# Autodesk Inventor assembly: Main Assembly
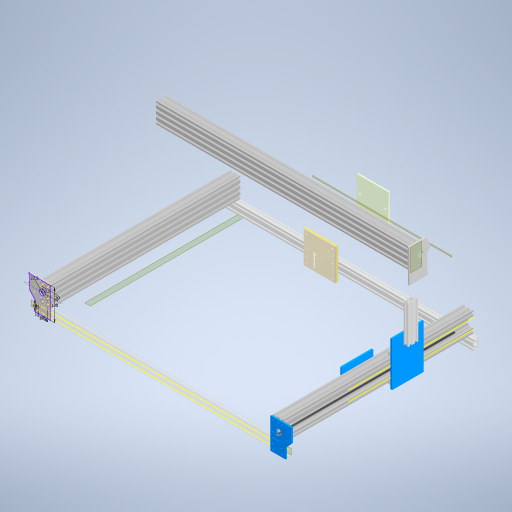
[picture p0: Inventor's stored thumbnail of the model, 512x512]
Saved by Autodesk Inventor 2023.2 (Build 272271000, 271)
## iProperties
Created: 2023-01-31
Part Number: Main Assembly
Document SubType Name: Assembly
Designer: dmargari
Mass: 176937 g
Surface Area: 89724.7 cm^2
Volume: 174359 cm^3
Density: 1.01479 g/cm^3
Author: dmargari
## iProperties of the stored document Solid-V-Xtreme-Wheel.ipt
Created: 2015-07-29
Part Number: Xtreme Solid V Wheel
Material: Generic
Description: STEP AP203
Document SubType Name: Modeling
Designer: dmargari
Density: 1 g/cm^3
Appearance: Default
Mass: 2.24603 g
Surface Area: 16.605 cm^2
Volume: 2.24603 cm^3
Sending System: SolidWorks 2014
Preprocessor: SwSTEP 2.0
Title: Xtreme Solid V Wheel.step
Revision Number: ANY
## iProperties of the stored document ACME-Nut-Block.ipt
Created: 2015-07-29
Part Number: 8mm Acme Nut Block
Material: Generic
Description: STEP AP203
Document SubType Name: Modeling
Designer: dmargari
Density: 1 g/cm^3
Appearance: Default
Sending System: SolidWorks 2014
Preprocessor: SwSTEP 2.0
Title: 8mm Acme Nut Block.step
Revision Number: ANY
## Documents named in this file (18)
- \\icnas3.cc.ic.ac.uk\dmargari\Inventor\Autosampler V3\Main Assembly.iam
- \\icnas3.cc.ic.ac.uk\dmargari\Inventor\Autosampler V3\Desk.ipt
- **\\icnas3.cc.ic.ac.uk\dmargari\Inventor\Autosampler V3\Main Assembly.iam*LocalDocs*xAaaaaibaAaaaaaaaAaaaapz5Ha*Solid-V-Xtreme-Wheel.ipt
- \\icnas3.cc.ic.ac.uk\dmargari\Inventor\Autosampler V3\C beam gantry (small side y axis).ipt
- \\icnas3.cc.ic.ac.uk\dmargari\Inventor\Autosampler V3\C beam gantry (big side y axis).ipt
- \\icnas3.cc.ic.ac.uk\dmargari\Inventor\Content Center Files\R2023\en-US\20x40\1000.ipt
- \\icnas3.cc.ic.ac.uk\dmargari\Inventor\Content Center Files\R2023\en-US\C beam extrusion\250.ipt
- **\\icnas3.cc.ic.ac.uk\dmargari\Inventor\Autosampler V3\Main Assembly.iam*LocalDocs*xAaaaaqaaAaaaaaaaAaaaqjz0Qe*ACME-Nut-Block.ipt
- \\icnas3.cc.ic.ac.uk\dmargari\Inventor\Autosampler V3\lead screw 8mm 700mm.ipt
- \\icnas3.cc.ic.ac.uk\dmargari\Inventor\Autosampler V3\Y axis motor mount new.ipt
- \\icnas3.cc.ic.ac.uk\dmargari\Inventor\Autosampler V3\X axis motor mount.ipt
- \\icnas3.cc.ic.ac.uk\dmargari\Inventor\Autosampler V3\20x40 extrusion x axis.ipt
- \\icnas3.cc.ic.ac.uk\dmargari\Inventor\Content Center Files\R2023\en-US\C beam extrusion\500.ipt
- \\icnas3.cc.ic.ac.uk\dmargari\Inventor\Autosampler V3\X axis carriage.ipt
- \\icnas3.cc.ic.ac.uk\dmargari\Inventor\Autosampler V3\X axis carriage small.ipt
- \\icnas3.cc.ic.ac.uk\dmargari\Inventor\Autosampler V3\X axis carriage small side.ipt
- \\icnas3.cc.ic.ac.uk\dmargari\Inventor\Autosampler V3\3rd-party-models\Solid-V-Xtreme-Wheel\Solid-V-Xtreme-Wheel.step
- \\icnas3.cc.ic.ac.uk\dmargari\Inventor\Autosampler V3\3rd-party-models\Ooznest-ACME-Nut-Block\ACME-Nut-Block.step
## Components (20 placed, 15 different names)
1. Desk:1 — Flush:2, Mate:31, Flush:44, Flush:45, Mate:32, Flush:47
2. C beam extrusion 250:1
3. C beam extrusion 250:2 — Flush:57
4. C beam gantry (small side y axis):1
5. C beam gantry (big side y axis):1 — Flush:57, Mate:34, Flush:50, Mate:35, Flush:51, Flush:52, Flush:58, Mate:42, Rigid:23
6. 20x40 extrusion x axis:1 — Mate:42, Rigid:23, Mate:43
7. 20x40 1000:1 — Mate:31, Flush:44, Flush:45, Mate:33, Mate:38, Flush:55, Flush:56
8. 20x40 1000:2 — Mate:32, Flush:47, Mate:33
9. ACME-Nut-Block:1 — Mate:34, Flush:50, Flush:58
10. ACME-Nut-Block:2 — Mate:35, Flush:51, Flush:52, Mate:36
11. lead screw 8mm 700mm:1 — Mate:36
12. Y axis motor mount new:1
13. Y axis motor mount new:2 — Mate:38, Flush:55, Flush:56
14. Solid-V-Xtreme-Wheel:9
15. Solid-V-Xtreme-Wheel:10
16. X axis motor mount:1 — Rotational:11, Mate:43
17. C beam extrusion 500:1 — Rotational:11
18. X axis carriage big:1
19. Z axis carriage small:1 — Flush:59
20. X axis carriage small:1 — Flush:59
## Relationships (32: Flush 17, Mate 13, WeldJoint 1, RevoluteJoint 1)
- Flush:2: Desk:1
- [Mate] (40 mm): Desk:1 ↔ C beam extrusion 250:1
- [Flush] (20 mm): Desk:1 ↔ C beam extrusion 250:1
- [Flush]: Desk:1 ↔ C beam extrusion 250:1
- [Mate] (40 mm): Desk:1 ↔ C beam extrusion 250:2
- [Flush]: Desk:1 ↔ C beam extrusion 250:2
- Flush:57 (-22 mm): C beam extrusion 250:2 ↔ C beam gantry (big side y axis):1
- [Mate] (25 mm): C beam extrusion 250:2 ↔ C beam gantry (big side y axis):1
- [Mate] (-30 mm): C beam extrusion 250:2 ↔ C beam gantry (small side y axis):1
- [Flush] (-20 mm): C beam extrusion 250:2 ↔ C beam gantry (small side y axis):1
- Mate:31: Desk:1 ↔ 20x40 1000:1
- Flush:44: Desk:1 ↔ 20x40 1000:1
- Flush:45: Desk:1 ↔ 20x40 1000:1
- [Flush] (20 mm): C beam extrusion 250:2 ↔ 20x40 1000:1
- Mate:32: Desk:1 ↔ 20x40 1000:2
- Flush:47: Desk:1 ↔ 20x40 1000:2
- Mate:33 (710 mm): 20x40 1000:1 ↔ 20x40 1000:2
- Mate:34: C beam gantry (big side y axis):1 ↔ ACME-Nut-Block:1
- Flush:50 (20 mm): C beam gantry (big side y axis):1 ↔ ACME-Nut-Block:1
- Mate:35: C beam gantry (big side y axis):1 ↔ ACME-Nut-Block:2
- Flush:51 (45 mm): C beam gantry (big side y axis):1 ↔ ACME-Nut-Block:2
- Flush:52 (20 mm): C beam gantry (big side y axis):1 ↔ ACME-Nut-Block:2
- Mate:36: ACME-Nut-Block:2 ↔ lead screw 8mm 700mm:1
- Mate:38: 20x40 1000:1 ↔ Y axis motor mount new:2
- Flush:55: 20x40 1000:1 ↔ Y axis motor mount new:2
- Flush:56: 20x40 1000:1 ↔ Y axis motor mount new:2
- Flush:58 (45 mm): C beam gantry (big side y axis):1 ↔ ACME-Nut-Block:1
- Mate:42: C beam gantry (big side y axis):1 ↔ 20x40 extrusion x axis:1
- Rigid:23 [WeldJoint]: C beam gantry (big side y axis):1 ↔ 20x40 extrusion x axis:1
- Rotational:11 [RevoluteJoint]: X axis motor mount:1 ↔ C beam extrusion 500:1
- Mate:43: 20x40 extrusion x axis:1 ↔ X axis motor mount:1
- Flush:59: Z axis carriage small:1 ↔ X axis carriage small:1
